# Autodesk Inventor assembly: ASY TKS 3590 FDS one way
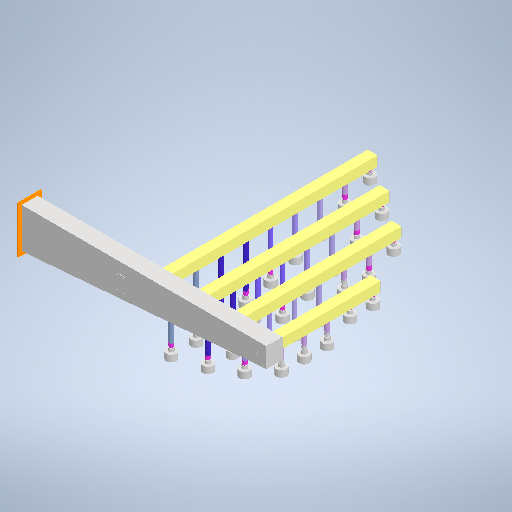
[picture p0: Inventor's stored thumbnail of the model, 512x512]
Saved by Autodesk Inventor 2025 (Build 290162010, 162A)
## iProperties
Created: 2025-07-22
Part Number: ASY TKS 3590 FDS one way
Document SubType Name: Assembly
Designer: admin
Stock Number: 20x40
Author: admin
## Documents named in this file (10)
- C:\Users\pokla\Documents\Inventor\ANP--Antipayuta\FDS 1400\ASY TKS 3590 FDS one way.iam
- C:\Users\pokla\Documents\Inventor\ANP--Antipayuta\FDS 1400\ANP 1422 BOTTOM FDS diameter way up.ipt
- C:\Users\pokla\Documents\Inventor\ANP--Antipayuta\FDS 1400\ANP 1421 FDS Diam way flange 1.ipt
- C:\Users\pokla\Documents\Inventor\ANP--Antipayuta\FDS 1400\ANP 1423 BOTTOM FDS diameter way down.ipt
- C:\Users\pokla\Documents\Inventor\ANP--Antipayuta\FDS 1400\ASY ANP 1424 FDS way 4.iam
- C:\Users\pokla\Documents\Inventor\ANP--Antipayuta\FDS 1400\ASY ANP 1425 FDS way 5.iam
- C:\Users\pokla\Documents\Inventor\ANP--Antipayuta\FDS 1400\ASY ANP 1426 FDS way 6.iam
- C:\Users\pokla\Documents\Inventor\ANP--Antipayuta\FDS 1400\ASY ANP 1427 FDS way 7.iam
- C:\Users\pokla\Documents\Inventor\ANP--Antipayuta\FDS 1400\ANP 1434 BOTTOM FDS support flange.ipt
- C:\Users\pokla\Documents\Inventor\ANP--Antipayuta\FDS 1400\ANP 1424 FDS diam way cup.ipt
## Components (9 placed, 9 different names)
1. TKS 3522 BOTTOM FDS diameter way up:1 — Rigid:11, Rigid:12, Rigid:13, Rigid:14
2. TKS 3521 BOTTOM FDS Diam way flange 1:1
3. TKS 3523 BOTTOM FDS diameter way down:1 — Rigid:16, Rigid:18
4. ASY TKS 3524 FDS way 4:1 [sub-assembly] — Rigid:11
5. ASY TKS 3525 FDS way 5:1 [sub-assembly] — Rigid:12
6. ASY TKS 3526 FDS way 6:1 [sub-assembly] — Rigid:13
7. ASY TKS 3527 FDS way 7:1 [sub-assembly] — Rigid:14
8. TKS 3561 BOTTOM FDS support flange:1 — Rigid:16
9. TKS 3524 FDS diam way cup:1 — Rigid:18
## Relationships (12: WeldJoint 6, Mate 3, Flush 3)
- [Mate]: TKS 3522 BOTTOM FDS diameter way up:1 ↔ TKS 3521 BOTTOM FDS Diam way flange 1:1
- [Flush]: TKS 3522 BOTTOM FDS diameter way up:1 ↔ TKS 3521 BOTTOM FDS Diam way flange 1:1
- [Flush]: TKS 3522 BOTTOM FDS diameter way up:1 ↔ TKS 3521 BOTTOM FDS Diam way flange 1:1
- [Mate]: TKS 3521 BOTTOM FDS Diam way flange 1:1 ↔ TKS 3523 BOTTOM FDS diameter way down:1
- [Flush]: TKS 3521 BOTTOM FDS Diam way flange 1:1 ↔ TKS 3523 BOTTOM FDS diameter way down:1
- [Mate]: TKS 3522 BOTTOM FDS diameter way up:1 ↔ TKS 3523 BOTTOM FDS diameter way down:1
- Rigid:11 [WeldJoint]: TKS 3522 BOTTOM FDS diameter way up:1 ↔ ASY TKS 3524 FDS way 4:1
- Rigid:12 [WeldJoint]: TKS 3522 BOTTOM FDS diameter way up:1 ↔ ASY TKS 3525 FDS way 5:1
- Rigid:13 [WeldJoint]: TKS 3522 BOTTOM FDS diameter way up:1 ↔ ASY TKS 3526 FDS way 6:1
- Rigid:14 [WeldJoint]: TKS 3522 BOTTOM FDS diameter way up:1 ↔ ASY TKS 3527 FDS way 7:1
- Rigid:16 [WeldJoint]: TKS 3523 BOTTOM FDS diameter way down:1 ↔ TKS 3561 BOTTOM FDS support flange:1
- Rigid:18 [WeldJoint]: TKS 3523 BOTTOM FDS diameter way down:1 ↔ TKS 3524 FDS diam way cup:1
